# Autodesk Inventor assembly: ChassisComplete_NERDS
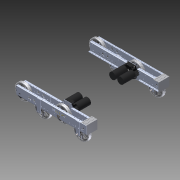
[picture p0: Inventor's stored thumbnail of the model, 180x180]
Saved by Autodesk Inventor 2014 (Build 180170000, 170)
## iProperties
Created: 2016-01-19
Part Number: ChassisComplete_NERDS
Document SubType Name: Assembly
Designer: choices
Author: choices
## Documents named in this file (12)
- Z:\Nerds_1726\Robot\Chassis\ChassisComplete_NERDS.iam
- Z:\Nerds_1726\AndyMark_Parts\6 HiGrip with hub and double pulley.iam
- Z:\Nerds_1726\AndyMark_Parts\FR8ZZ Hex Bearing.ipt
- Z:\Nerds_1726\AndyMark_Parts\am-2598_107 2016 KOP Toughbox Mini.iam
- Z:\Nerds_1726\AndyMark_Parts\6 HiGrip with bearings, pulleys and spacers.iam
- Z:\Nerds_1726\Robot\Chassis\Chass_InsideSheetTabs.ipt
- Z:\Nerds_1726\AndyMark_Parts\375-16 x 4.25 Hex Bolt_HFBOLT 0.375-16x2.5x1-C.ipt
- Z:\Nerds_1726\Robot\Chassis\Chassis_OutsideSheetCustom.ipt
- Z:\Nerds_1726\Robot\Chassis\Chassis_OutsideSheetCustomLeft.ipt
- Z:\Nerds_1726\Robot\Chassis\Chass_InsideSheetTabsLeft.ipt
- Z:\Nerds_1726\Robot\Chassis\Chass_EndCaps.ipt
- Z:\Nerds_1726\Robot\Chassis\Chassis_Motor.ipt
## Components (24 placed, 11 different names)
1. 6 HiGrip with hub and double pulley:1 [sub-assembly] — Mate:7, Mate:8, Mate:9
2. am-2598_107 2016 KOP Toughbox Mini:1 [sub-assembly] — Mate:8, Mate:9, Mate:12, Mate:14, Flush:1, Mate:15, Mate:16, Mate:17, Insert:19, Insert:20
3. FR8ZZ Hex Bearing:1 — Mate:7, Mate:12, Mate:14, Flush:1, Mate:18, Mate:19
4. 6 HiGrip with bearings, pulleys and spacers:1 [sub-assembly] — Insert:5, Tangent:1
5. Chass_InsideSheetTabs:1 — Mate:15, Mate:16, Mate:17, Insert:5, Insert:6, Insert:8, Flush:2
6. 6 HiGrip with bearings, pulleys and spacers:2 [sub-assembly] — Insert:6
7. 6 HiGrip with bearings, pulleys and spacers:4 [sub-assembly] — Insert:8
8. Chassis_OutsideSheetCustom:1 — Mate:18, Mate:19, Insert:9, Flush:3, Mate:29, Mate:31, Mate:32
9. 375-16 x 4.25 Hex Bolt_HFBOLT 0.375-16x2.5x1-C:1 — Insert:9, Tangent:1
10. Chassis_OutsideSheetCustomLeft:1 — Insert:12, Insert:13, Insert:15, Flush:3, Mate:27, Mate:28, Mate:33
11. Chass_InsideSheetTabsLeft:1 — Mate:26, Insert:10, Insert:11, Insert:14, Insert:16, Flush:2
12. 6 HiGrip with hub and double pulley:2 [sub-assembly] — Mate:20, Mate:21, Mate:22, Mate:23
13. 6 HiGrip with bearings, pulleys and spacers:5 [sub-assembly] — Insert:13, Tangent:2
14. 6 HiGrip with bearings, pulleys and spacers:6 [sub-assembly] — Insert:15
15. 6 HiGrip with bearings, pulleys and spacers:7 [sub-assembly] — Insert:16
16. am-2598_107 2016 KOP Toughbox Mini:2 [sub-assembly] — Mate:20, Mate:21, Mate:22, Mate:24, Mate:25, Mate:26, Insert:10, Insert:11, Insert:17, Insert:18
17. FR8ZZ Hex Bearing:2 — Mate:23, Mate:24, Mate:25, Insert:12
18. 375-16 x 4.25 Hex Bolt_HFBOLT 0.375-16x2.5x1-C:2 — Insert:14, Tangent:2
19. Chass_EndCaps:1 — Mate:29, Mate:31, Mate:32
20. Chass_EndCaps:2 — Mate:27, Mate:28, Mate:33
21. Chassis_Motor:1 — Insert:17
22. Chassis_Motor:2 — Insert:20
23. Chassis_Motor:3 — Insert:18
24. Chassis_Motor:4 — Insert:19
## Relationships (43: Mate 23, Insert 15, Flush 3, Tangent 2)
- Mate:7: 6 HiGrip with hub and double pulley:1 ↔ FR8ZZ Hex Bearing:1
- Mate:8: 6 HiGrip with hub and double pulley:1 ↔ am-2598_107 2016 KOP Toughbox Mini:1
- Mate:9: 6 HiGrip with hub and double pulley:1 ↔ am-2598_107 2016 KOP Toughbox Mini:1
- Mate:12: am-2598_107 2016 KOP Toughbox Mini:1 ↔ FR8ZZ Hex Bearing:1
- Mate:14: am-2598_107 2016 KOP Toughbox Mini:1 ↔ FR8ZZ Hex Bearing:1
- Flush:1: am-2598_107 2016 KOP Toughbox Mini:1 ↔ FR8ZZ Hex Bearing:1
- Mate:15: am-2598_107 2016 KOP Toughbox Mini:1 ↔ Chass_InsideSheetTabs:1
- Mate:16: am-2598_107 2016 KOP Toughbox Mini:1 ↔ Chass_InsideSheetTabs:1
- Mate:17: am-2598_107 2016 KOP Toughbox Mini:1 ↔ Chass_InsideSheetTabs:1
- Insert:5: 6 HiGrip with bearings, pulleys and spacers:1 ↔ Chass_InsideSheetTabs:1
- Insert:6: Chass_InsideSheetTabs:1 ↔ 6 HiGrip with bearings, pulleys and spacers:2
- Insert:8: Chass_InsideSheetTabs:1 ↔ 6 HiGrip with bearings, pulleys and spacers:4
- Mate:18: FR8ZZ Hex Bearing:1 ↔ Chassis_OutsideSheetCustom:1
- Mate:19: FR8ZZ Hex Bearing:1 ↔ Chassis_OutsideSheetCustom:1
- Insert:9: Chassis_OutsideSheetCustom:1 ↔ 375-16 x 4.25 Hex Bolt_HFBOLT 0.375-16x2.5x1-C:1
- Tangent:1: 6 HiGrip with bearings, pulleys and spacers:1 ↔ 375-16 x 4.25 Hex Bolt_HFBOLT 0.375-16x2.5x1-C:1
- Mate:20: 6 HiGrip with hub and double pulley:2 ↔ am-2598_107 2016 KOP Toughbox Mini:2
- Mate:21: 6 HiGrip with hub and double pulley:2 ↔ am-2598_107 2016 KOP Toughbox Mini:2
- Mate:22: 6 HiGrip with hub and double pulley:2 ↔ am-2598_107 2016 KOP Toughbox Mini:2
- Mate:23: 6 HiGrip with hub and double pulley:2 ↔ FR8ZZ Hex Bearing:2
- Mate:24: am-2598_107 2016 KOP Toughbox Mini:2 ↔ FR8ZZ Hex Bearing:2
- Mate:25: am-2598_107 2016 KOP Toughbox Mini:2 ↔ FR8ZZ Hex Bearing:2
- Mate:26: Chass_InsideSheetTabsLeft:1 ↔ am-2598_107 2016 KOP Toughbox Mini:2
- Insert:10: Chass_InsideSheetTabsLeft:1 ↔ am-2598_107 2016 KOP Toughbox Mini:2
- Insert:11: Chass_InsideSheetTabsLeft:1 ↔ am-2598_107 2016 KOP Toughbox Mini:2
- Insert:12: Chassis_OutsideSheetCustomLeft:1 ↔ FR8ZZ Hex Bearing:2
- Insert:13: Chassis_OutsideSheetCustomLeft:1 ↔ 6 HiGrip with bearings, pulleys and spacers:5
- Insert:14: Chass_InsideSheetTabsLeft:1 ↔ 375-16 x 4.25 Hex Bolt_HFBOLT 0.375-16x2.5x1-C:2
- Tangent:2: 6 HiGrip with bearings, pulleys and spacers:5 ↔ 375-16 x 4.25 Hex Bolt_HFBOLT 0.375-16x2.5x1-C:2
- Insert:15: Chassis_OutsideSheetCustomLeft:1 ↔ 6 HiGrip with bearings, pulleys and spacers:6
- Insert:16: Chass_InsideSheetTabsLeft:1 ↔ 6 HiGrip with bearings, pulleys and spacers:7
- Flush:2: Chass_InsideSheetTabs:1 ↔ Chass_InsideSheetTabsLeft:1
- Flush:3: Chassis_OutsideSheetCustom:1 ↔ Chassis_OutsideSheetCustomLeft:1
- Mate:27: Chassis_OutsideSheetCustomLeft:1 ↔ Chass_EndCaps:2
- Mate:28: Chassis_OutsideSheetCustomLeft:1 ↔ Chass_EndCaps:2
- Mate:29: Chassis_OutsideSheetCustom:1 ↔ Chass_EndCaps:1
- Insert:17: am-2598_107 2016 KOP Toughbox Mini:2 ↔ Chassis_Motor:1
- Insert:18: am-2598_107 2016 KOP Toughbox Mini:2 ↔ Chassis_Motor:3
- Insert:19: am-2598_107 2016 KOP Toughbox Mini:1 ↔ Chassis_Motor:4
- Insert:20: am-2598_107 2016 KOP Toughbox Mini:1 ↔ Chassis_Motor:2
- Mate:31: Chassis_OutsideSheetCustom:1 ↔ Chass_EndCaps:1
- Mate:32: Chassis_OutsideSheetCustom:1 ↔ Chass_EndCaps:1
- Mate:33: Chassis_OutsideSheetCustomLeft:1 ↔ Chass_EndCaps:2
